# Autodesk Inventor assembly: BaseMotor1
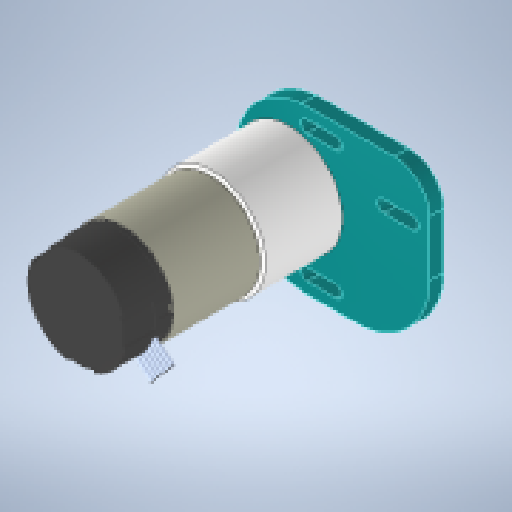
[picture p0: Inventor's stored thumbnail of the model, 512x512]
Saved by Autodesk Inventor 2024.3 (Build 283343000, 343)
## iProperties
Created: 2024-09-30
Part Number: BaseMotor1
Document SubType Name: Assembly
Designer: User
Author: User
## Documents named in this file (3)
- C:\Users\User\Documents\Universidad Octavo Semestre\Robotica Industrial\matlab\SCARA\mariana_scara_final\mariana_scara_final\BaseMotor1.iam
- C:\Users\User\Documents\Universidad Octavo Semestre\Robotica Industrial\matlab\SCARA\mariana_scara_final\mariana_scara_final\lamina_motor_superior.ipt
- C:\Users\User\Documents\Universidad Octavo Semestre\Robotica Industrial\matlab\SCARA\mariana_scara_final\mariana_scara_final\motor_1.ipt
## Components (2 placed, 2 different names)
1. lamina_motor_superior:1 — Insert:1
2. motor_1:1 — Insert:1
## Relationships (1: Insert 1)
- Insert:1: lamina_motor_superior:1 ↔ motor_1:1
